# Autodesk Inventor assembly: Soyuz Assembly
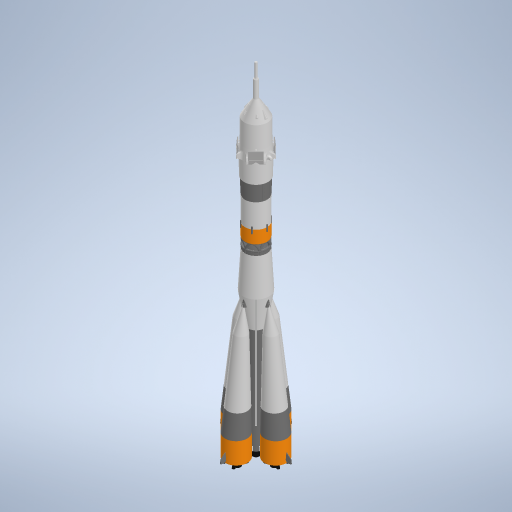
[picture p0: Inventor's stored thumbnail of the model, 512x512]
Saved by Autodesk Inventor 2023 (Build 270158030, 158C)
## iProperties
Created: 2023-01-06
Part Number: Soyuz Assembly
Document SubType Name: Assembly
Designer: Imogen Heard
Author: Imogen Heard
## Documents named in this file (11)
- C:\Users\dheard\Documents\Inventor\Inventor_Projects\Soyuz Model\Soyuz Assembly.iam
- C:\Users\dheard\Documents\Inventor\Inventor_Projects\Soyuz Model\Stage2 Core Booster.ipt
- C:\Users\dheard\Documents\Inventor\Inventor_Projects\Soyuz Model\Interstage1.ipt
- C:\Users\dheard\Documents\Inventor\Inventor_Projects\Soyuz Model\Stage 1 Booster.ipt
- C:\Users\dheard\Documents\Inventor\Inventor_Projects\Soyuz Model\Interstage 2.ipt
- C:\Users\dheard\Documents\Inventor\Inventor_Projects\Soyuz Model\3rd Stage.ipt
- C:\Users\dheard\Documents\Inventor\Inventor_Projects\Soyuz Model\3rd Stage Part B.ipt
- C:\Users\dheard\Documents\Inventor\Inventor_Projects\Soyuz Model\Fairing.ipt
- C:\Users\dheard\Documents\Inventor\Inventor_Projects\Soyuz Model\Core Booster Part B.ipt
- C:\Users\dheard\Documents\Inventor\Inventor_Projects\Soyuz Model\Grid Fins.ipt
- C:\Users\dheard\Documents\Inventor\Inventor_Projects\Soyuz Model\Escape Tower.ipt
## Components (17 placed, 10 different names)
1. Stage2 Core Booster:1 — Insert:1, Insert:2, Insert:3, Insert:4
2. Core Booster Part B:1
3. Interstage1:1 — Insert:5
4. Stage 1 Booster:1 — Insert:1
5. Stage 1 Booster:2 — Insert:2
6. Stage 1 Booster:3 — Insert:3
7. Stage 1 Booster:4 — Insert:4
8. Interstage 2:1 — Insert:5, Insert:6
9. 3rd Stage:1 — Insert:6, Insert:7
10. 3rd Stage Part B:1 — Insert:7, Insert:8, Insert:9
11. Fairing:1 — Insert:8, Rotational:1, Rotational:3
12. Fairing:2 — Insert:9, Rotational:4, Rotational:5, Insert:10
13. Grid Fins:1 — Rotational:1
14. Grid Fins:2 — Rotational:4
15. Grid Fins:3 — Rotational:3
16. Grid Fins:4 — Rotational:5
17. Escape Tower:1 — Insert:10
## Relationships (14: Insert 10, RevoluteJoint 4)
- Insert:1: Stage2 Core Booster:1 ↔ Stage 1 Booster:1
- Insert:2: Stage2 Core Booster:1 ↔ Stage 1 Booster:2
- Insert:3: Stage2 Core Booster:1 ↔ Stage 1 Booster:3
- Insert:4: Stage2 Core Booster:1 ↔ Stage 1 Booster:4
- Insert:5 (-1.4 mm): Interstage1:1 ↔ Interstage 2:1
- Insert:6: Interstage 2:1 ↔ 3rd Stage:1
- Insert:7: 3rd Stage:1 ↔ 3rd Stage Part B:1
- Insert:8 (1.4 mm): 3rd Stage Part B:1 ↔ Fairing:1
- Insert:9: 3rd Stage Part B:1 ↔ Fairing:2
- Rotational:1 [RevoluteJoint]: Fairing:1 ↔ Grid Fins:1
- Rotational:3 [RevoluteJoint]: Fairing:1 ↔ Grid Fins:3
- Rotational:4 [RevoluteJoint]: Fairing:2 ↔ Grid Fins:2
- Rotational:5 [RevoluteJoint]: Fairing:2 ↔ Grid Fins:4
- Insert:10: Fairing:2 ↔ Escape Tower:1
